# Autodesk Inventor assembly: Intake Assembly
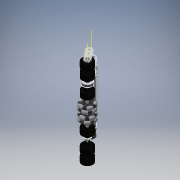
[picture p0: Inventor's stored thumbnail of the model, 180x180]
Saved by Autodesk Inventor 2019.4 (Build 234330000, 330)
## iProperties
Created: 2020-01-28
Part Number: Intake Assembly
Document SubType Name: Assembly
Designer: admin
Mass: 2152.42 g
Surface Area: 4846.19 cm^2
Volume: 1170.44 cm^3
Density: 1.83898 g/cm^3
Author: admin
## Documents named in this file (16)
- C:\Users\admin\Desktop\FRC 2020 Engineering\GitHub\7738-2020\Robot V2\Intake V2\Intake Assembly.iam
- C:\Users\admin\Desktop\FRC 2020 Engineering\GitHub\7738-2020\Robot V2\Intake V2\Intake Arm.ipt
- C:\Users\admin\Desktop\FRC 2020 Engineering\GitHub\7738-2020\Robot V2\Intake V2\Omni Wheel\3_25_Omni-Directional_Wheel_217-4775.iam
- C:\Users\admin\Desktop\FRC 2020 Engineering\GitHub\7738-2020\Robot V2\Intake V2\Intake Assembly\Design Accelerator\Synchronous Belts Transmission1.iam
- C:\Users\admin\Desktop\FRC 2020 Engineering\GitHub\7738-2020\Robot V2\Intake System\MF148ZZ.ipt
- C:\Users\admin\Desktop\FRC 2020 Engineering\GitHub\7738-2020\Robot V2\Turret\F6800.ipt
- C:\Users\admin\Desktop\FRC 2020 Engineering\GitHub\7738-2020\Robot V2\Intake V2\Saftey Axle.ipt
- C:\Users\admin\Desktop\FRC 2020 Engineering\GitHub\7738-2020\Robot V2\Intake V2\Intake Plate Spacer.ipt
- C:\Users\admin\Desktop\FRC 2020 Engineering\GitHub\7738-2020\Robot V2\Intake V2\Intake Axle.ipt
- C:\Users\admin\Desktop\FRC 2020 Engineering\GitHub\7738-2020\Robot V2\Intake V2\Pneumatic Spcaer.ipt
- C:\Users\admin\Desktop\FRC 2020 Engineering\GitHub\7738-2020\Robot V2\Intake V2\60mm Mecanum Wheel.ipt
- C:\Users\admin\Desktop\FRC 2020 Engineering\GitHub\7738-2020\Storage system\Protection Plates.ipt
- C:\Users\admin\Desktop\FRC 2020 Engineering\GitHub\7738-2020\Storage system\F608.ipt
- C:\Users\admin\Desktop\FRC 2020 Engineering\GitHub\7738-2020\Storage system\118 mm Spacer.ipt
- C:\Users\admin\Desktop\FRC 2020 Engineering\GitHub\7738-2020\Robot V2\Intake V2\30t_Aluminum_Spur_Gear_20_DP_3_8_Hex_Bore_217-3210.ipt
- C:\Users\admin\Desktop\FRC 2020 Engineering\GitHub\7738-2020\Robot V2\Intake V2\775pro_775pro_Connect_and_8T_Pinion_217-6459.ipt
## Components (32 placed, 15 different names)
1. Intake Arm:1 — Mate:1, Mate:2, Mate:3, Mate:4, Mate:6, Mate:7, Mate:11, Mate:13, Mate:15, Mate:18, Mate:60, Mate:61, Mate:108, Mate:109, Mate:110, Mate:119, Mate:120, Mate:121, Mate:122, Mate:124, Mate:125, Mate:128, Mate:134
2. Intake Arm:2 — Mate:1, Mate:2, Mate:3, Mate:8, Mate:16, Mate:17, Mate:21, Mate:22, Mate:55, Mate:56, Mate:57, Mate:58, Mate:59, Mate:62, Mate:91, Mate:92, Mate:105, Mate:106, Mate:107, Mate:115, Mate:116, Mate:117, Mate:118, Mate:133
3. 3_25_Omni-Directional_Wheel_217-4775:1 [sub-assembly] — Mate:4, Mate:134
4. 3_25_Omni-Directional_Wheel_217-4775:3 [sub-assembly] — Mate:6, Mate:133
5. Synchronous Belts Transmission:1 [sub-assembly]
6. MF148ZZ:2 — Mate:11, Mate:13, Mate:53
7. F6800:1 — Mate:15, Mate:18
8. F6800:2 — Mate:16, Mate:17
9. MF148ZZ:4 — Mate:21, Mate:22, Mate:123
10. Saftey Axle:1 — Mate:53, Mate:123, Mate:126, Mate:127
11. Intake Plate Spacer:1 — Mate:55, Mate:57
12. Intake Plate Spacer:2 — Mate:56, Mate:58
13. F6800:3 — Mate:59, Mate:62, Mate:63, Mate:64, Flush:3, Mate:131
14. F6800:4 — Mate:60, Mate:61, Mate:132
15. Intake Axle:1 — Mate:63, Mate:64, Flush:2, Mate:101, Mate:102, Mate:103, Mate:129, Mate:130
16. Pneumatic Spcaer:1 — Mate:91, Mate:92
17. 60mm Mecanum Wheel:2 — Mate:93, Flush:3, Mate:100, Mate:101
18. 60mm Mecanum Wheel:3 — Mate:93, Mate:100
19. 60mm Mecanum Wheel:5 — Flush:2, Mate:99, Mate:102
20. 60mm Mecanum Wheel:6 — Mate:99, Mate:103
21. Protection Plates:1 — Mate:105, Mate:106, Mate:107, Mate:111, Mate:112
22. Protection Plates:2 — Mate:108, Mate:109, Mate:110, Mate:113, Mate:114
23. F608:1 — Mate:111, Mate:112
24. F608:2 — Mate:113, Mate:114
25. 118 mm Spacer:1 — Mate:115, Mate:116
26. 118 mm Spacer:2 — Mate:117, Mate:118
27. 118 mm Spacer:3 — Mate:119, Mate:120
28. 118 mm Spacer:4 — Mate:121, Mate:122
29. 30t_Aluminum_Spur_Gear_20_DP_3_8_Hex_Bore_217-3210:1 — Mate:126, Mate:127
30. 775pro_775pro_Connect_and_8T_Pinion_217-6459:1 — Mate:124, Mate:125, Mate:128
31. 60mm Mecanum Wheel:7 — Mate:129, Mate:131
32. 60mm Mecanum Wheel:8 — Mate:130, Mate:132
## Relationships (66: Mate 64, Flush 2)
- Mate:1: Intake Arm:1 ↔ Intake Arm:2
- Mate:2: Intake Arm:1 ↔ Intake Arm:2
- Mate:3 (248.6 mm): Intake Arm:1 ↔ Intake Arm:2
- Mate:4: Intake Arm:1 ↔ 3_25_Omni-Directional_Wheel_217-4775:1
- Mate:6: Intake Arm:1 ↔ 3_25_Omni-Directional_Wheel_217-4775:3
- Mate:7: Intake Arm:1
- Mate:8 (119.3 mm): Intake Arm:2
- Mate:11: Intake Arm:1 ↔ MF148ZZ:2
- Mate:13 (0.2 mm): Intake Arm:1 ↔ MF148ZZ:2
- Mate:15: Intake Arm:1 ↔ F6800:1
- Mate:16: Intake Arm:2 ↔ F6800:2
- Mate:17 (0.2 mm): Intake Arm:2 ↔ F6800:2
- Mate:18 (0.2 mm): Intake Arm:1 ↔ F6800:1
- Mate:21: Intake Arm:2 ↔ MF148ZZ:4
- Mate:22 (0.2 mm): Intake Arm:2 ↔ MF148ZZ:4
- Mate:53: MF148ZZ:2 ↔ Saftey Axle:1
- Mate:55: Intake Arm:2 ↔ Intake Plate Spacer:1
- Mate:56: Intake Arm:2 ↔ Intake Plate Spacer:2
- Mate:57: Intake Arm:2 ↔ Intake Plate Spacer:1
- Mate:58: Intake Arm:2 ↔ Intake Plate Spacer:2
- Mate:59: Intake Arm:2 ↔ F6800:3
- Mate:60: Intake Arm:1 ↔ F6800:4
- Mate:61 (0.2 mm): Intake Arm:1 ↔ F6800:4
- Mate:62 (0.2 mm): Intake Arm:2 ↔ F6800:3
- Mate:63: F6800:3 ↔ Intake Axle:1
- Mate:64 (60 mm): F6800:3 ↔ Intake Axle:1
- Mate:91: Intake Arm:2 ↔ Pneumatic Spcaer:1
- Mate:92: Intake Arm:2 ↔ Pneumatic Spcaer:1
- Mate:93: 60mm Mecanum Wheel:2 ↔ 60mm Mecanum Wheel:3
- Flush:2 (60 mm): Intake Axle:1 ↔ 60mm Mecanum Wheel:5
- Mate:99 (1.4 mm): 60mm Mecanum Wheel:5 ↔ 60mm Mecanum Wheel:6
- Flush:3 (25.1 mm): F6800:3 ↔ 60mm Mecanum Wheel:2
- Mate:100 (1.4 mm): 60mm Mecanum Wheel:2 ↔ 60mm Mecanum Wheel:3
- Mate:101: Intake Axle:1 ↔ 60mm Mecanum Wheel:2
- Mate:102: Intake Axle:1 ↔ 60mm Mecanum Wheel:5
- Mate:103: Intake Axle:1 ↔ 60mm Mecanum Wheel:6
- Mate:105 (118 mm): Intake Arm:2 ↔ Protection Plates:1
- Mate:106: Intake Arm:2 ↔ Protection Plates:1
- Mate:107: Intake Arm:2 ↔ Protection Plates:1
- Mate:108 (118 mm): Intake Arm:1 ↔ Protection Plates:2
- Mate:109: Intake Arm:1 ↔ Protection Plates:2
- Mate:110: Intake Arm:1 ↔ Protection Plates:2
- Mate:111: Protection Plates:1 ↔ F608:1
- Mate:112: Protection Plates:1 ↔ F608:1
- Mate:113: Protection Plates:2 ↔ F608:2
- Mate:114: Protection Plates:2 ↔ F608:2
- Mate:115: Intake Arm:2 ↔ 118 mm Spacer:1
- Mate:116: Intake Arm:2 ↔ 118 mm Spacer:1
- Mate:117: Intake Arm:2 ↔ 118 mm Spacer:2
- Mate:118: Intake Arm:2 ↔ 118 mm Spacer:2
- Mate:119: Intake Arm:1 ↔ 118 mm Spacer:3
- Mate:120: Intake Arm:1 ↔ 118 mm Spacer:3
- Mate:121: Intake Arm:1 ↔ 118 mm Spacer:4
- Mate:122: Intake Arm:1 ↔ 118 mm Spacer:4
- Mate:123: MF148ZZ:4 ↔ Saftey Axle:1
- Mate:124: Intake Arm:1 ↔ 775pro_775pro_Connect_and_8T_Pinion_217-6459:1
- Mate:125: Intake Arm:1 ↔ 775pro_775pro_Connect_and_8T_Pinion_217-6459:1
- Mate:126: Saftey Axle:1 ↔ 30t_Aluminum_Spur_Gear_20_DP_3_8_Hex_Bore_217-3210:1
- Mate:127: Saftey Axle:1 ↔ 30t_Aluminum_Spur_Gear_20_DP_3_8_Hex_Bore_217-3210:1
- Mate:128: Intake Arm:1 ↔ 775pro_775pro_Connect_and_8T_Pinion_217-6459:1
- Mate:129: Intake Axle:1 ↔ 60mm Mecanum Wheel:7
- Mate:130: Intake Axle:1 ↔ 60mm Mecanum Wheel:8
- Mate:131 (1 mm): F6800:3 ↔ 60mm Mecanum Wheel:7
- Mate:132 (1 mm): F6800:4 ↔ 60mm Mecanum Wheel:8
- Mate:133 (80 mm): Intake Arm:2 ↔ 3_25_Omni-Directional_Wheel_217-4775:3
- Mate:134 (80 mm): Intake Arm:1 ↔ 3_25_Omni-Directional_Wheel_217-4775:1
